# Autodesk Inventor assembly: bed bracket right
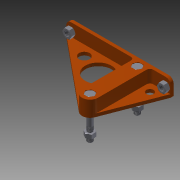
[picture p0: Inventor's stored thumbnail of the model, 180x180]
Saved by Autodesk Inventor 2013 (Build 170138000, 138)
## iProperties
Created: 2013-10-14
Part Number: bed bracket right
Document SubType Name: Assembly
Designer: employee
Author: employee
## Documents named in this file (5)
- C:\Users\employee\Desktop\new wally\bed bracket right.iam
- C:\Users\employee\Desktop\new wally\bed bracket right.ipt
- C:\Users\employee\Desktop\new wally\M8 nut.ipt
- C:\Users\employee\Desktop\new wally\M8x60.ipt
- C:\Users\employee\Desktop\new wally\washer.ipt
## Components (9 placed, 4 different names)
1. bed bracket right:1 — Insert:1, Insert:2, Angle:1, Angle:2, Insert:3, Insert:4, Insert:5, Insert:6
2. Hex Nut Metric M8 x 1.25:1 — Insert:3
3. Hex Nut Metric M8 x 1.25:2 — Insert:4
4. Hex Nut Metric M8 x 1.25:3 — Insert:7
5. Hex Nut Metric M8 x 1.25:4 — Insert:8
6. Hex Bolt - Metric M8 x 1.25 x 60:1 — Insert:1, Angle:1
7. Hex Bolt - Metric M8 x 1.25 x 60:2 — Insert:2, Angle:2
8. washer:1 — Insert:5, Insert:7
9. washer:2 — Insert:6, Insert:8
## Relationships (10: Insert 8, Angle 2)
- Insert:1: bed bracket right:1 ↔ Hex Bolt - Metric M8 x 1.25 x 60:1
- Insert:2: bed bracket right:1 ↔ Hex Bolt - Metric M8 x 1.25 x 60:2
- Angle:1 (0 deg): bed bracket right:1 ↔ Hex Bolt - Metric M8 x 1.25 x 60:1
- Angle:2 (0 deg): bed bracket right:1 ↔ Hex Bolt - Metric M8 x 1.25 x 60:2
- Insert:3: bed bracket right:1 ↔ Hex Nut Metric M8 x 1.25:1
- Insert:4: bed bracket right:1 ↔ Hex Nut Metric M8 x 1.25:2
- Insert:5: bed bracket right:1 ↔ washer:1
- Insert:6: bed bracket right:1 ↔ washer:2
- Insert:7 (25 mm): Hex Nut Metric M8 x 1.25:3 ↔ washer:1
- Insert:8 (25 mm): Hex Nut Metric M8 x 1.25:4 ↔ washer:2
